# Autodesk Inventor assembly: aircilinder_30
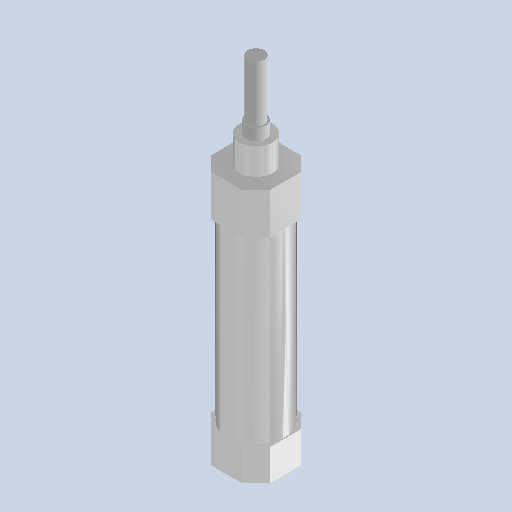
[picture p0: Inventor's stored thumbnail of the model, 512x512]
Saved by Autodesk Inventor 2025.1 (Build 291241000, 241)
## iProperties
Created: 2022-08-24
Part Number: aircilinder_30
Document SubType Name: Assembly
Designer: zegi
Mass: 50.236 g
Surface Area: 76.9659 cm^2
Volume: 19.5282 cm^3
Density: 2.57249 g/cm^3
Author: zegi
## Documents named in this file (3)
- C:\Users\haruy\Documents\ロボコン\NHK2025\cad\000_parts\エアシリンダー\airclinder\aircilinder_30.iam
- C:\Users\haruy\Documents\ロボコン\NHK2025\cad\000_parts\エアシリンダー\airclinder\aircilinder_30_lod.ipt
- C:\Users\haruy\Documents\ロボコン\NHK2025\cad\000_parts\エアシリンダー\airclinder\airclinder_30.ipt
## Components (2 placed, 2 different names)
1. aircilinder_30_lod:1 — 円柱状:1
2. airclinder_30:1 — 円柱状:1
## Relationships (1: CylindricalJoint 1)
- 円柱状:1 [CylindricalJoint]: aircilinder_30_lod:1 ↔ airclinder_30:1
